# Autodesk Inventor assembly: 大粗轴锁轴器螺丝螺帽套
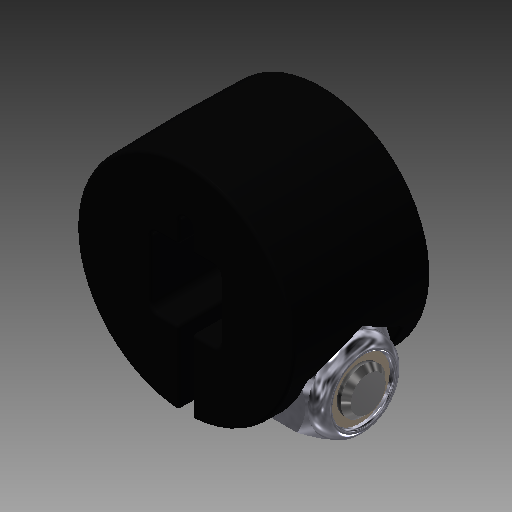
[picture p0: Inventor's stored thumbnail of the model, 512x512]
Saved by Autodesk Inventor 2019.3 (Build 233278000, 278)
## iProperties
Created: 2019-03-26
Part Number: 大粗轴锁轴器螺丝螺帽套
Material: 常规
Document SubType Name: Assembly
Designer: aresp
Mass: 27.3798 g
Surface Area: 25.6777 cm^2
Volume: 3.49463 cm^3
Density: 7.83481 g/cm^3
Author: aresp
## Documents named in this file (4)
- D:\cad\零件库\大粗轴锁轴器螺丝螺帽套.iam
- D:\cad\零件库\轴\Lock Collar HS (plastic).ipt
- D:\cad\零件库\螺丝螺帽\Nut 8-32 Nylock.ipt
- D:\cad\零件库\螺丝螺帽\Screw 8-32 x 0.625'' - Black.ipt
## Components (3 placed, 3 different names)
1. Lock Collar HS (plastic):1
2. Nut 8-32 Nylock:1
3. Screw 8-32 x 0.625'' - Black:1
## Relationships (4: Mate 4)
- [Mate]: Lock Collar HS (plastic):1 ↔ Screw 8-32 x 0.625'' - Black:1
- [Mate]: Lock Collar HS (plastic):1 ↔ Screw 8-32 x 0.625'' - Black:1
- [Mate]: Lock Collar HS (plastic):1 ↔ Nut 8-32 Nylock:1
- [Mate]: Nut 8-32 Nylock:1 ↔ Screw 8-32 x 0.625'' - Black:1
